# Autodesk Inventor assembly: подшипник
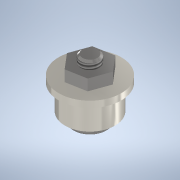
[picture p0: Inventor's stored thumbnail of the model, 180x180]
Saved by Autodesk Inventor 2020.1 (Build 241239000, 239)
## iProperties
Created: 2021-08-12
Part Number: подшипник
Document SubType Name: Assembly
Designer: User
Author: User
## Documents named in this file (4)
- D:\GitHub\avatar-kvantoriada\3D\подшипник.iam
- C:\Users\User\Documents\Inventor\Content Center Files\R2020\ru-RU\AS 1474(1)\AS 1474 - M3(1).ipt
- C:\Users\User\Documents\Inventor\Content Center Files\R2020\ru-RU\AS 1427(08)\AS 1427 - M3 x 8(6) I.ipt
- D:\GitHub\avatar-kvantoriada\3D\подшипник.ipt
## Components (3 placed, 3 different names)
1. AS 1427 Z - метрическая M3 x 8:10 — Жесткий:12
2. подшипник:1 — Жесткий:11, Жесткий:12
3. AS 1474 - метрическая M3:6 — Жесткий:11
## Relationships (2: WeldJoint 2)
- Жесткий:11 [WeldJoint]: подшипник:1 ↔ AS 1474 - метрическая M3:6
- Жесткий:12 [WeldJoint]: AS 1427 Z - метрическая M3 x 8:10 ↔ подшипник:1
